# Autodesk Inventor assembly: PMT_Adaptor
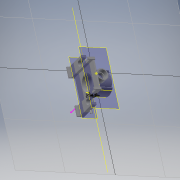
[picture p0: Inventor's stored thumbnail of the model, 180x180]
Saved by Autodesk Inventor 2016 (Build 200138000, 138)
## iProperties
Created: 2016-05-10
Part Number: PMT_Adaptor
Document SubType Name: Assembly
Designer: pupa
Author: pupa
## Documents named in this file (5)
- D:\Machine\PMT_Adaptor_ver3\PMT_Adaptor.iam
- D:\Machine\PMT_Adaptor_ver3\PMT_ADAPTOR.ipt
- D:\Machine\PMT_Adaptor_ver3\PMT_Adaptor_Shutter.ipt
- D:\Machine\PMT_Adaptor_ver3\PMT_VialBase.ipt
- D:\Machine\PMT_Adaptor_ver3\PMT_Ring.ipt
## Components (4 placed, 4 different names)
1. PMT_ADAPTOR:1 — Mate:2, Mate:3, Angle:1, Slider:1, Flush:1, Flush:2
2. Shutter:1 — Mate:2, Mate:3, Angle:1, Slider:1
3. PMT_VialBase:1 — Flush:1, Flush:2, Flush:3
4. PMT_Ring:1 — Flush:4
## Relationships (8: Flush 4, Mate 2, Angle 1, TranslationJoint 1)
- Mate:2: PMT_ADAPTOR:1 ↔ Shutter:1
- Mate:3: PMT_ADAPTOR:1 ↔ Shutter:1
- Angle:1 (0 deg): PMT_ADAPTOR:1 ↔ Shutter:1
- Slider:1 [TranslationJoint]: PMT_ADAPTOR:1 ↔ Shutter:1
- Flush:1: PMT_ADAPTOR:1 ↔ PMT_VialBase:1
- Flush:2 (85 mm): PMT_ADAPTOR:1 ↔ PMT_VialBase:1
- Flush:3 (40 mm): PMT_VialBase:1
- Flush:4: PMT_Ring:1
